# Autodesk Inventor assembly: A600 Keyboard
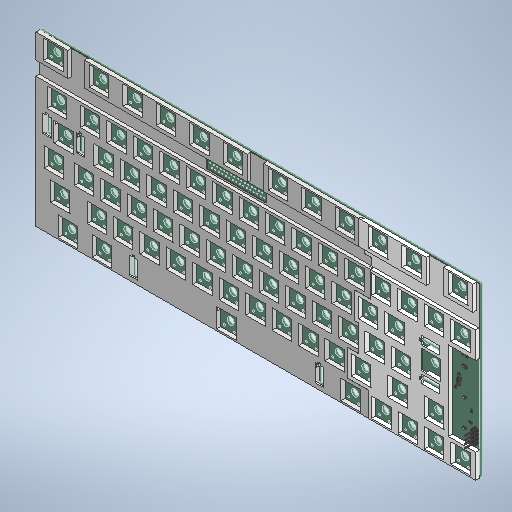
[picture p0: Inventor's stored thumbnail of the model, 512x512]
Saved by Autodesk Inventor 2025 (Build 290162000, 162)
## iProperties
Created: 2024-08-15
Part Number: A600 Keyboard
Document SubType Name: Assembly
Designer: adam
Author: adam
## Documents named in this file (4)
- C:\Users\adam\Projects\A600KBv2\3dprint\Keyboard Plates\A600 Keyboard.iam
- C:\Users\adam\Projects\A600KBv2\3dprint\Keyboard Plates\A600KBv3\A600KBv3.ipt
- C:\Users\adam\Projects\A600KBv2\3dprint\Keyboard Plates\Left Plate.ipt
- C:\Users\adam\Projects\A600KBv2\3dprint\Keyboard Plates\Right Plate.ipt
## Components (3 placed, 3 different names)
1. A600KBv3:1 — Flush:1, Flush:2
2. Left Plate:1 — Flush:1
3. Right Plate:1 — Flush:2
## Relationships (2: Flush 2)
- Flush:1: A600KBv3:1 ↔ Left Plate:1
- Flush:2: A600KBv3:1 ↔ Right Plate:1
